# Autodesk Inventor assembly: back_brace
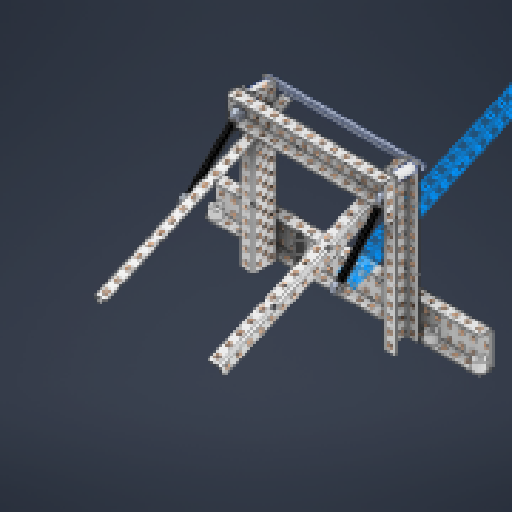
[picture p0: Inventor's stored thumbnail of the model, 512x512]
Saved by Autodesk Inventor 2024 (Build 280153000, 153)
## iProperties
Created: 2023-10-19
Part Number: back_brace
Document SubType Name: Assembly
Designer: avere
Author: avere
## Documents named in this file (7)
- D:\vex_robotics\hardware\cad\goated_v0.1\chassis\back_brace.iam
- D:\vex_robotics\hardware\cad\VEX-CAD-Inventor-1.41\Motion\Spacers\Spacer Nylon .500 OD\NSpacer White .500 OD x .375.ipt
- D:\vex_robotics\hardware\cad\goated_v0.1\catapult\tower.iam
- D:\vex_robotics\hardware\cad\VEX-CAD-Inventor-1.41\Motion\Spacers\Spacer Nylon .500 OD.ipt
- D:\vex_robotics\hardware\cad\VEX-CAD-Inventor-1.41\Structure\Angle\Aluminum 1x1\Alu Angle 1x1x17.ipt
- D:\vex_robotics\hardware\cad\VEX-CAD-Inventor-1.41\Structure\C Channel\Aluminum 1x3x1\Alu C 1x3x1x25.ipt
- D:\vex_robotics\hardware\cad\VEX-CAD-Inventor-1.41\Structure\C Channel\Aluminum 1x2x1\Alu C 1x2x1x12.ipt
## Components (9 placed, 5 different names)
1. tower:1 [sub-assembly] — Insert:15, Insert:21, Mate:4, Insert:22, Mate:5
2. Alu Angle 1x1x17:1 — Insert:24, Mate:7
3. Alu Angle 1x1x17:2 — Insert:15, Insert:23, Mate:6
4. Alu C 1x3x1x25:1 — Insert:17, Insert:18, Insert:19, Insert:20, Insert:21, Mate:4, Insert:22, Mate:5
5. NSpacer White .500 OD x .375:5 — Insert:17
6. NSpacer White .500 OD x .375:6 — Insert:18
7. NSpacer White .500 OD x .375:7 — Insert:20
8. NSpacer White .500 OD x .375:8 — Insert:19
9. Alu C 1x2x1x12:1 — Insert:23, Mate:6, Insert:24, Mate:7
## Relationships (13: Insert 9, Mate 4)
- Insert:15 (1.5875 mm): tower:1 ↔ Alu Angle 1x1x17:2
- Insert:17: Alu C 1x3x1x25:1 ↔ NSpacer White .500 OD x .375:5
- Insert:18: Alu C 1x3x1x25:1 ↔ NSpacer White .500 OD x .375:6
- Insert:19: Alu C 1x3x1x25:1 ↔ NSpacer White .500 OD x .375:8
- Insert:20: Alu C 1x3x1x25:1 ↔ NSpacer White .500 OD x .375:7
- Insert:21 (12.7 mm): tower:1 ↔ Alu C 1x3x1x25:1
- Mate:4: tower:1 ↔ Alu C 1x3x1x25:1
- Insert:22 (12.7 mm): tower:1 ↔ Alu C 1x3x1x25:1
- Mate:5: tower:1 ↔ Alu C 1x3x1x25:1
- Insert:23: Alu Angle 1x1x17:2 ↔ Alu C 1x2x1x12:1
- Mate:6: Alu Angle 1x1x17:2 ↔ Alu C 1x2x1x12:1
- Insert:24: Alu Angle 1x1x17:1 ↔ Alu C 1x2x1x12:1
- Mate:7: Alu Angle 1x1x17:1 ↔ Alu C 1x2x1x12:1
